# Autodesk Inventor assembly: Mockup Assembly
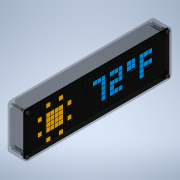
[picture p0: Inventor's stored thumbnail of the model, 180x180]
Saved by Autodesk Inventor 2020 (Build 240168000, 168)
## iProperties
Created: 2021-04-14
Part Number: Mockup Assembly
Document SubType Name: Assembly
Designer: user
Author: user
## Documents named in this file (7)
- C:\Users\user\OneDrive - UW\Projects\Pixel Weather\Inventor Parts\Mockup Assembly.iam
- C:\Users\user\OneDrive - UW\Projects\Pixel Weather\Inventor Parts\Case Full.ipt
- C:\Users\user\OneDrive - UW\Projects\Pixel Weather\Inventor Parts\Acrylic Front Plate.ipt
- C:\Users\user\OneDrive - UW\Projects\Pixel Weather\Inventor Parts\Grid Full.ipt
- C:\Users\user\OneDrive - UW\Projects\Pixel Weather\Inventor Parts\Current Temp Mockup.ipt
- C:\Users\user\OneDrive - UW\Projects\Pixel Weather\Inventor Parts\Sun Icon Mockup.ipt
- C:\Users\user\OneDrive - UW\Projects\Pixel Weather\Inventor Parts\M5 Cap Head Screw.ipt
## Components (9 placed, 6 different names)
1. Case Full:1 — Mate:1, Mate:2, Mate:3
2. Acrylic Front Plate:1 — Mate:4, Mate:5, Mate:6, Mate:11, Mate:12, Mate:13, Mate:14, Mate:15, Mate:16, Mate:17, Mate:18
3. Grid Full:1 — Mate:1, Mate:2, Mate:3, Mate:4, Mate:5, Mate:6, Mate:7, Mate:8, Flush:1, Mate:9, Mate:10, Flush:2
4. Current Temp Mockup:1 — Mate:9, Mate:10, Flush:2
5. Sun Icon Mockup:1 — Mate:7, Mate:8, Flush:1
6. M5 Cap Head Screw:2 — Mate:11, Mate:12
7. M5 Cap Head Screw:3 — Mate:13, Mate:14
8. M5 Cap Head Screw:4 — Mate:16, Mate:18
9. M5 Cap Head Screw:5 — Mate:15, Mate:17
## Relationships (20: Mate 18, Flush 2)
- Mate:1: Case Full:1 ↔ Grid Full:1
- Mate:2: Case Full:1 ↔ Grid Full:1
- Mate:3: Case Full:1 ↔ Grid Full:1
- Mate:4: Acrylic Front Plate:1 ↔ Grid Full:1
- Mate:5: Acrylic Front Plate:1 ↔ Grid Full:1
- Mate:6: Acrylic Front Plate:1 ↔ Grid Full:1
- Mate:7: Grid Full:1 ↔ Sun Icon Mockup:1
- Mate:8: Grid Full:1 ↔ Sun Icon Mockup:1
- Flush:1 (-3.01 mm): Grid Full:1 ↔ Sun Icon Mockup:1
- Mate:9: Grid Full:1 ↔ Current Temp Mockup:1
- Mate:10: Grid Full:1 ↔ Current Temp Mockup:1
- Flush:2 (-3.01 mm): Grid Full:1 ↔ Current Temp Mockup:1
- Mate:11: Acrylic Front Plate:1 ↔ M5 Cap Head Screw:2
- Mate:12: Acrylic Front Plate:1 ↔ M5 Cap Head Screw:2
- Mate:13: Acrylic Front Plate:1 ↔ M5 Cap Head Screw:3
- Mate:14: Acrylic Front Plate:1 ↔ M5 Cap Head Screw:3
- Mate:15: Acrylic Front Plate:1 ↔ M5 Cap Head Screw:5
- Mate:16: Acrylic Front Plate:1 ↔ M5 Cap Head Screw:4
- Mate:17: Acrylic Front Plate:1 ↔ M5 Cap Head Screw:5
- Mate:18: Acrylic Front Plate:1 ↔ M5 Cap Head Screw:4
